# Autodesk Inventor assembly: MainAssembly
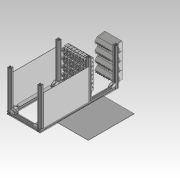
[picture p0: Inventor's stored thumbnail of the model, 180x180]
Saved by Autodesk Inventor 2020 (Build 240168000, 168)
## iProperties
Created: 2021-09-11
Part Number: MainAssembly
Document SubType Name: Assembly
Designer: DDeGo
Author: DDeGo
## Documents named in this file (11)
- C:\Users\DDeGo\Documents\Drew\Projects\Gravity-Holo-Display\cad\MainAssembly.iam
- C:\Users\DDeGo\Documents\Drew\Projects\Gravity-Holo-Display\cad\SolenoidRack.iam
- C:\Users\DDeGo\Documents\Drew\Projects\Gravity-Holo-Display\cad\Panel.ipt
- C:\Users\DDeGo\Documents\Drew\Projects\Gravity-Holo-Display\cad\Extrusion 250mm.ipt
- C:\Users\DDeGo\Documents\Drew\Projects\Gravity-Holo-Display\cad\Extrusion Corner Bracket.ipt
- C:\Users\DDeGo\Documents\Drew\Projects\Gravity-Holo-Display\cad\LedBracket.ipt
- C:\Users\DDeGo\Documents\Drew\Projects\Gravity-Holo-Display\cad\Extrusion 300mm.ipt
- C:\Users\DDeGo\Documents\Drew\Projects\Gravity-Holo-Display\cad\NozzleAligner.ipt
- C:\Users\DDeGo\Documents\Drew\Projects\Gravity-Holo-Display\cad\Extrusion 180mm.ipt
- C:\Users\DDeGo\Documents\Drew\Projects\Gravity-Holo-Display\cad\Tank_8output.ipt
- C:\Users\DDeGo\Documents\Drew\Projects\Gravity-Holo-Display\cad\DoubleSolenoidRack.iam
## Components (40 placed, 10 different names)
1. Extrusion 250mm:1 — Flush:1, Mate:5, Angle:1, Mate:8, Flush:3, Flush:9, Mate:14, Mate:17, Mate:38, Mate:47
2. Extrusion 250mm:2 — Flush:1, Mate:6, Mate:7, Flush:4, Flush:6, Mate:13, Mate:15, Flush:25, Mate:30, Mate:33, Mate:58, Mate:59, Angle:2
3. Panel:1
4. Panel:2 — Mate:7, Flush:4, Flush:5
5. Panel:3 — Mate:8, Flush:3, Flush:5
6. Extrusion 300mm:1 — Flush:9, Flush:13, Mate:16, Flush:15, Mate:22, Flush:16, Mate:23, Flush:18, Mate:36, Flush:29, Mate:43, Flush:32, Flush:35, Mate:47, Flush:37, Flush:38, Mate:48, Flush:39
7. Extrusion 300mm:2 — Flush:6, Flush:10, Mate:18, Flush:14, Mate:21, Flush:17, Mate:24, Flush:19, Mate:28, Mate:31, Flush:27, Mate:45, Flush:33, Flush:34, Flush:36, Mate:49, Mate:53, Flush:40, Mate:55, Flush:42
8. Extrusion 250mm:5 — Flush:10, Mate:20, Flush:22, Mate:29, Mate:39, Mate:49
9. Extrusion 250mm:6 — Flush:13, Mate:19, Mate:41, Mate:48, Flush:39
10. Extrusion Corner Bracket:1 — Mate:15, Mate:18, Flush:14
11. Extrusion Corner Bracket:2 — Mate:16, Mate:17, Flush:15
12. Extrusion Corner Bracket:3 — Mate:20, Mate:21, Flush:17, Mate:25
13. Extrusion Corner Bracket:4 — Mate:19, Mate:22, Flush:16
14. LedBracket:1 — Mate:24, Flush:19, Flush:20, Mate:25
15. LedBracket:2 — Mate:23, Flush:18, Flush:20
16. NozzleAligner:1
17. Extrusion 180mm:1 — Flush:22, Mate:29, Mate:40, Mate:42, Flush:30, Flush:31, Mate:44, Mate:46, Flush:36, Flush:37, Flush:38, Mate:50, Mate:51, Mate:52, Mate:60
18. Extrusion 180mm:2 — Flush:25, Mate:30, Mate:32, Flush:26, Mate:34, Mate:35, Mate:37, Flush:28, Flush:34, Flush:35, Mate:60
19. Extrusion Corner Bracket:5 — Mate:37, Mate:38, Flush:28
20. Extrusion Corner Bracket:6 — Mate:32, Mate:33, Flush:26
21. Extrusion Corner Bracket:7 — Mate:35, Mate:36, Flush:29
22. Extrusion Corner Bracket:8 — Mate:31, Flush:27, Mate:34
23. Extrusion Corner Bracket:9 — Mate:39, Mate:42, Flush:30
24. Extrusion Corner Bracket:10 — Mate:40, Mate:41, Flush:31
25. Extrusion Corner Bracket:11 — Mate:43, Mate:44, Flush:32
26. Extrusion Corner Bracket:12 — Mate:45, Mate:46, Flush:33
27. Extrusion 250mm:7 — Mate:54, Flush:41, Mate:55, Flush:42, Mate:56, Flush:43
28. Extrusion Corner Bracket:13 — Mate:53, Mate:54, Flush:40, Flush:41
29. SolenoidRack:4 [sub-assembly] — Mate:5, Angle:1, Mate:6, Mate:14
30. SolenoidRack:5 [sub-assembly]
31. SolenoidRack:6 [sub-assembly]
32. SolenoidRack:7 [sub-assembly] — Mate:13, Mate:28
33. Tank_8output:1 — Mate:56, Flush:43
34. Tank_8output:2
35. Tank_8output:3
36. Tank_8output:4
37. DoubleSolenoidRack:1 [sub-assembly] — Mate:58, Mate:59, Angle:2
38. DoubleSolenoidRack:2 [sub-assembly]
39. DoubleSolenoidRack:3 [sub-assembly]
40. DoubleSolenoidRack:4 [sub-assembly]
## Component patterns: (4 elements, first: SolenoidRack:4), (4 elements, first: Tank_8output:1), (4 elements, first: DoubleSolenoidRack:1)
## Relationships (86: Mate 49, Flush 35, Angle 2)
- Flush:1: Extrusion 250mm:1 ↔ Extrusion 250mm:2
- Mate:5 (-10 mm): Extrusion 250mm:1 ↔ SolenoidRack:4
- Angle:1 (0 deg): Extrusion 250mm:1 ↔ SolenoidRack:4
- Mate:6 (-10 mm): Extrusion 250mm:2 ↔ SolenoidRack:4
- Mate:7: Extrusion 250mm:2 ↔ Panel:2
- Mate:8: Extrusion 250mm:1 ↔ Panel:3
- Flush:3: Extrusion 250mm:1 ↔ Panel:3
- Flush:4: Extrusion 250mm:2 ↔ Panel:2
- Flush:5: Panel:2 ↔ Panel:3
- Flush:6: Extrusion 250mm:2 ↔ Extrusion 300mm:2
- Flush:9: Extrusion 250mm:1 ↔ Extrusion 300mm:1
- Flush:10: Extrusion 300mm:2 ↔ Extrusion 250mm:5
- Flush:13: Extrusion 300mm:1 ↔ Extrusion 250mm:6
- Mate:13: Extrusion 250mm:2 ↔ SolenoidRack:7
- Mate:14: Extrusion 250mm:1 ↔ SolenoidRack:4
- Mate:15: Extrusion 250mm:2 ↔ Extrusion Corner Bracket:1
- Mate:16: Extrusion 300mm:1 ↔ Extrusion Corner Bracket:2
- Mate:17: Extrusion 250mm:1 ↔ Extrusion Corner Bracket:2
- Mate:18: Extrusion 300mm:2 ↔ Extrusion Corner Bracket:1
- Flush:14: Extrusion 300mm:2 ↔ Extrusion Corner Bracket:1
- Flush:15: Extrusion 300mm:1 ↔ Extrusion Corner Bracket:2
- Mate:19: Extrusion 250mm:6 ↔ Extrusion Corner Bracket:4
- Mate:20: Extrusion 250mm:5 ↔ Extrusion Corner Bracket:3
- Mate:21: Extrusion 300mm:2 ↔ Extrusion Corner Bracket:3
- Mate:22: Extrusion 300mm:1 ↔ Extrusion Corner Bracket:4
- Flush:16: Extrusion 300mm:1 ↔ Extrusion Corner Bracket:4
- Flush:17: Extrusion 300mm:2 ↔ Extrusion Corner Bracket:3
- Mate:23: Extrusion 300mm:1 ↔ LedBracket:2
- Mate:24: Extrusion 300mm:2 ↔ LedBracket:1
- Flush:18: Extrusion 300mm:1 ↔ LedBracket:2
- Flush:19: Extrusion 300mm:2 ↔ LedBracket:1
- Flush:20: LedBracket:1 ↔ LedBracket:2
- Mate:25 (2 mm): Extrusion Corner Bracket:3 ↔ LedBracket:1
- Mate:28 (25 mm): Extrusion 300mm:2 ↔ SolenoidRack:7
- Flush:22: Extrusion 250mm:5 ↔ Extrusion 180mm:1
- Mate:29: Extrusion 250mm:5 ↔ Extrusion 180mm:1
- Flush:25: Extrusion 250mm:2 ↔ Extrusion 180mm:2
- Mate:30: Extrusion 250mm:2 ↔ Extrusion 180mm:2
- Mate:31: Extrusion 300mm:2 ↔ Extrusion Corner Bracket:8
- Mate:32: Extrusion 180mm:2 ↔ Extrusion Corner Bracket:6
- Mate:33: Extrusion 250mm:2 ↔ Extrusion Corner Bracket:6
- Flush:26: Extrusion 180mm:2 ↔ Extrusion Corner Bracket:6
- Flush:27: Extrusion 300mm:2 ↔ Extrusion Corner Bracket:8
- Mate:34: Extrusion 180mm:2 ↔ Extrusion Corner Bracket:8
- Mate:35: Extrusion 180mm:2 ↔ Extrusion Corner Bracket:7
- Mate:36: Extrusion 300mm:1 ↔ Extrusion Corner Bracket:7
- Mate:37: Extrusion 180mm:2 ↔ Extrusion Corner Bracket:5
- Mate:38: Extrusion 250mm:1 ↔ Extrusion Corner Bracket:5
- Flush:28: Extrusion 180mm:2 ↔ Extrusion Corner Bracket:5
- Flush:29: Extrusion 300mm:1 ↔ Extrusion Corner Bracket:7
- Mate:39: Extrusion 250mm:5 ↔ Extrusion Corner Bracket:9
- Mate:40: Extrusion 180mm:1 ↔ Extrusion Corner Bracket:10
- Mate:41: Extrusion 250mm:6 ↔ Extrusion Corner Bracket:10
- Mate:42: Extrusion 180mm:1 ↔ Extrusion Corner Bracket:9
- Flush:30: Extrusion 180mm:1 ↔ Extrusion Corner Bracket:9
- Flush:31: Extrusion 180mm:1 ↔ Extrusion Corner Bracket:10
- Mate:43: Extrusion 300mm:1 ↔ Extrusion Corner Bracket:11
- Mate:44: Extrusion 180mm:1 ↔ Extrusion Corner Bracket:11
- Flush:32: Extrusion 300mm:1 ↔ Extrusion Corner Bracket:11
- Mate:45: Extrusion 300mm:2 ↔ Extrusion Corner Bracket:12
- Mate:46: Extrusion 180mm:1 ↔ Extrusion Corner Bracket:12
- Flush:33: Extrusion 300mm:2 ↔ Extrusion Corner Bracket:12
- Flush:34: Extrusion 300mm:2 ↔ Extrusion 180mm:2
- Flush:35: Extrusion 300mm:1 ↔ Extrusion 180mm:2
- Mate:47: Extrusion 250mm:1 ↔ Extrusion 300mm:1
- Flush:36: Extrusion 300mm:2 ↔ Extrusion 180mm:1
- Flush:37: Extrusion 300mm:1 ↔ Extrusion 180mm:1
- Flush:38: Extrusion 300mm:1 ↔ Extrusion 180mm:1
- Mate:48: Extrusion 300mm:1 ↔ Extrusion 250mm:6
- Flush:39: Extrusion 300mm:1 ↔ Extrusion 250mm:6
- Mate:49: Extrusion 300mm:2 ↔ Extrusion 250mm:5
- Mate:50: Extrusion 180mm:1
- Mate:51: Extrusion 180mm:1
- Mate:52: Extrusion 180mm:1
- Mate:53: Extrusion 300mm:2 ↔ Extrusion Corner Bracket:13
- Mate:54: Extrusion 250mm:7 ↔ Extrusion Corner Bracket:13
- Flush:40: Extrusion 300mm:2 ↔ Extrusion Corner Bracket:13
- Flush:41: Extrusion 250mm:7 ↔ Extrusion Corner Bracket:13
- Mate:55: Extrusion 300mm:2 ↔ Extrusion 250mm:7
- Flush:42: Extrusion 300mm:2 ↔ Extrusion 250mm:7
- Mate:56: Extrusion 250mm:7 ↔ Tank_8output:1
- Flush:43: Extrusion 250mm:7 ↔ Tank_8output:1
- Mate:58: Extrusion 250mm:2 ↔ DoubleSolenoidRack:1
- Mate:59 (-10 mm): Extrusion 250mm:2 ↔ DoubleSolenoidRack:1
- Mate:60 (300 mm): Extrusion 180mm:1 ↔ Extrusion 180mm:2
- Angle:2 (0 deg): Extrusion 250mm:2 ↔ DoubleSolenoidRack:1
